# Autodesk Inventor assembly: Sheathing_For_Roof
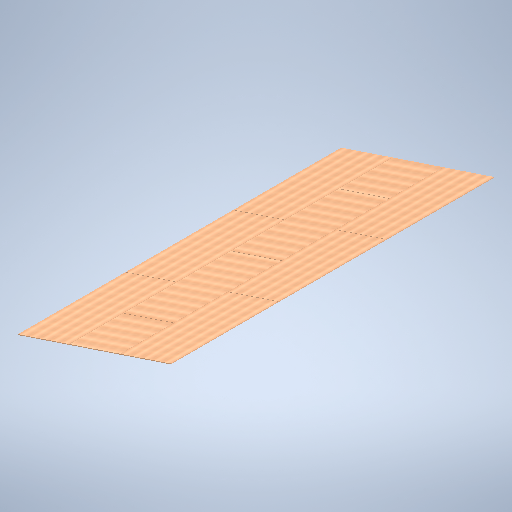
[picture p0: Inventor's stored thumbnail of the model, 512x512]
Saved by Autodesk Inventor 2025 (Build 290162010, 162A)
## iProperties
Created: 2024-10-03
Part Number: Sheathing_For_Roof
Document SubType Name: Assembly
Designer: Tom
Author: Tom
## Documents named in this file (5)
- C:\Users\Tom\Documents\Inventor\Mobility\Additional_Building\Sheathing_For_Roof.iam
- C:\Users\Tom\Documents\Inventor\Mobility\Additional_Building\OSB_For_Rear_Roof.ipt
- C:\Users\Tom\Documents\Inventor\Mobility\Additional_Building\OSB_For_Roof_With_Dimensions_48_x_48.ipt
- C:\Users\Tom\Documents\Inventor\Mobility\Additional_Building\OSB_For_Roof_With_Dimensions_48_x_96.ipt
- C:\Users\Tom\Documents\Inventor\Mobility\Additional_Building\OSB_For_Front_Roof.ipt
## Components (10 placed, 4 different names)
1. OSB_For_Rear_Roof:1 — Mate:1, Flush:1, Flush:2, Flush:3
2. OSB_For_Rear_Roof:2 — Mate:2
3. OSB_For_Rear_Roof:3
4. OSB_For_Roof_With_Dimensions_48_x_96:1 — Mate:2, Flush:3, Mate:3, Flush:4
5. OSB_For_Roof_With_Dimensions_48_x_96:2
6. OSB_For_Roof_With_Dimensions_48_x_48:1 — Mate:1, Flush:1, Flush:2, Mate:3, Mate:4, Flush:5
7. OSB_For_Roof_With_Dimensions_48_x_48:2
8. OSB_For_Front_Roof:1 — Mate:4, Flush:4, Flush:5
9. OSB_For_Front_Roof:2
10. OSB_For_Front_Roof:3
## Component patterns: (3 elements, first: OSB_For_Rear_Roof:1), (2 elements, first: OSB_For_Roof_With_Dimensions_48_x_96:1), (2 elements, first: OSB_For_Roof_With_Dimensions_48_x_48:1), (3 elements, first: OSB_For_Front_Roof:1)
## Relationships (9: Flush 5, Mate 4)
- Mate:1: OSB_For_Rear_Roof:1 ↔ OSB_For_Roof_With_Dimensions_48_x_48:1
- Flush:1: OSB_For_Rear_Roof:1 ↔ OSB_For_Roof_With_Dimensions_48_x_48:1
- Flush:2: OSB_For_Rear_Roof:1 ↔ OSB_For_Roof_With_Dimensions_48_x_48:1
- Mate:2: OSB_For_Rear_Roof:2 ↔ OSB_For_Roof_With_Dimensions_48_x_96:1
- Flush:3: OSB_For_Rear_Roof:1 ↔ OSB_For_Roof_With_Dimensions_48_x_96:1
- Mate:3: OSB_For_Roof_With_Dimensions_48_x_96:1 ↔ OSB_For_Roof_With_Dimensions_48_x_48:1
- Mate:4: OSB_For_Roof_With_Dimensions_48_x_48:1 ↔ OSB_For_Front_Roof:1
- Flush:4: OSB_For_Roof_With_Dimensions_48_x_96:1 ↔ OSB_For_Front_Roof:1
- Flush:5: OSB_For_Roof_With_Dimensions_48_x_48:1 ↔ OSB_For_Front_Roof:1
